# Autodesk Inventor assembly: Assembly3
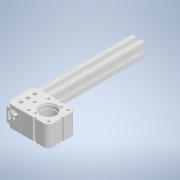
[picture p0: Inventor's stored thumbnail of the model, 180x180]
Saved by Autodesk Inventor 2020 (Build 240168000, 168)
## iProperties
Created: 2020-01-08
Part Number: Assembly3
Document SubType Name: Assembly
Designer: srini
Author: srini
## Documents named in this file (3)
- C:\Users\srini\Documents\FRC\2020\Assembly3.iam
- C:\Users\srini\Documents\FRC\2020\1003-9-CL.ipt
- C:\Users\srini\Documents\FRC\2020\SingleSideBearing.ipt
## Components (2 placed, 2 different names)
1. 1003-9-CL:1 — Flush:1
2. SingleSideBearing:1 — Flush:1
## Relationships (1: Flush 1)
- Flush:1: 1003-9-CL:1 ↔ SingleSideBearing:1
